# Autodesk Inventor assembly: YTP-AP-K01-R1.0
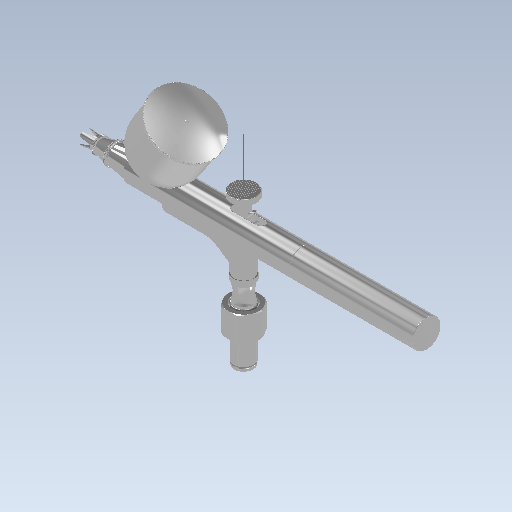
[picture p0: Inventor's stored thumbnail of the model, 512x512]
Saved by Autodesk Inventor 2020.4 (Build 244396000, 396)
## iProperties
RuleStatus: InUse
AfterDocNew0: iPropertyEnforcement
Created: 2021-08-29
Part Number: YTP-AP-K01-R1.0
Document SubType Name: Assembly
Designer: Uwe Wieser
Mass: 82.8737 g
Surface Area: 222.974 cm^2
Volume: 16.7279 cm^3
Density: 4.95421 g/cm^3
Project: Airbrush
Description: Iwata-HP-C-Airbrush
Author: Uwe Wieser
## Documents named in this file (23)
- F:\Autodesk-Inventor2020\YTP-Projekte\Airbrush\YTP-AP-K01-R1.0.iam
- F:\Autodesk-Inventor2020\YTP-Projekte\Airbrush\YTP-AP-E02-R1.0.ipt
- F:\Autodesk-Inventor2020\YTP-Projekte\Airbrush\YTP-AP-E03-R1.0.ipt
- F:\Autodesk-Inventor2020\YTP-Projekte\Airbrush\YTP-AP-E04-R1.0.ipt
- F:\Autodesk-Inventor2020\YTP-Projekte\Airbrush\YTP-AP-E05-R1.0.ipt
- F:\Autodesk-Inventor2020\YTP-Projekte\Airbrush\YTP-AP-E06-R1.0.ipt
- F:\Autodesk-Inventor2020\YTP-Projekte\Airbrush\YTP-AP-E07-R1.0.ipt
- F:\Autodesk-Inventor2020\YTP-Projekte\Airbrush\YTP-AP-E08-R1.0.ipt
- F:\Autodesk-Inventor2020\YTP-Projekte\Airbrush\YTP-AP-E09-R1.0.ipt
- F:\Autodesk-Inventor2020\YTP-Projekte\Airbrush\YTP-AP-E10-R1.0.ipt
- F:\Autodesk-Inventor2020\YTP-Projekte\Airbrush\YTP-AP-E11-R1.0.ipt
- F:\Autodesk-Inventor2020\YTP-Projekte\Airbrush\YTP-AP-E12-R1.0.ipt
- F:\Autodesk-Inventor2020\YTP-Projekte\Airbrush\YTP-AP-E13-R1.0.ipt
- F:\Autodesk-Inventor2020\YTP-Projekte\Airbrush\YTP-AP-E14-R1.0.ipt
- F:\Autodesk-Inventor2020\YTP-Projekte\Airbrush\YTP-AP-E15-R1.0.ipt
- F:\Autodesk-Inventor2020\YTP-Projekte\Airbrush\YTP-AP-E16-R1.0.ipt
- F:\Autodesk-Inventor2020\YTP-Projekte\Airbrush\YTP-AP-E17-R1.0.ipt
- F:\Autodesk-Inventor2020\YTP-Projekte\Airbrush\YTP-AP-E18-R1.0.ipt
- F:\Autodesk-Inventor2020\YTP-Projekte\Airbrush\YTP-AP-E19-R1.0.ipt
- F:\Autodesk-Inventor2020\YTP-Projekte\Airbrush\YTP-AP-E01-R1.1.ipt
- F:\Autodesk-Inventor2020\YTP-Projekte\Airbrush\YTP-AP-E20-R1.0.ipt
- F:\Autodesk-Inventor2020\YTP-Projekte\Airbrush\YTP-AP-E21-R1.0.ipt
- F:\Autodesk-Inventor2020\YTP-Projekte\Airbrush\YTP-AP-E22-R1.0.ipt
## Components (22 placed, 22 different names)
1. YTP-AP-E01-R1.1:1 — Passend:1, Fluchtend:1, Fluchtend:2, Einfügen:1, Passend:3, Tangential:1, Passend:4, Einfügen:2, Passend:6, Passend:7, Einfügen:5, Fluchtend:3, Einfügen:6, Fluchtend:4, Passend:16, Passend:17, Passend:20, Passend:27, Passend:28, Einfügen:7
2. YTP-AP-E02-R1.0:1 — Einfügen:2, Passend:7, Passend:19, Passend:21, Passend:25, Passend:30, Passend:31, Einfügen:9
3. YTP-AP-E03-R1.0:1 — Einfügen:1, Passend:29
4. YTP-AP-E04-R1.0:1 — Passend:2, Passend:3, Tangential:2
5. YTP-AP-E05-R1.0:1 — Passend:2, Tangential:1, Tangential:2
6. YTP-AP-E06-R1.0:1 — Passend:4, Passend:9, Passend:13, Passend:16
7. YTP-AP-E07-R1.0:1 — Einfügen:4, Passend:5, Passend:6, Einfügen:7
8. YTP-AP-E08-R1.0:1 — Einfügen:4, Passend:5
9. YTP-AP-E09-R1.0:1 — Einfügen:5, Passend:8
10. YTP-AP-E10-R1.0:1 — Fluchtend:3, Tangential:3, Passend:18, Tangential:4
11. YTP-AP-E11-R1.0:1 — Einfügen:6
12. YTP-AP-E12-R1.0:1 — Passend:9, Passend:10, Passend:11, Passend:12, Fluchtend:4
13. YTP-AP-E13-R1.0:1 — Passend:10, Passend:11, Passend:12, Passend:14, Winkel:1, Passend:15
14. YTP-AP-E14-R1.0:1 — Passend:13, Passend:14, Winkel:1, Passend:15, Passend:28, Einfügen:8
15. YTP-AP-E15-R1.0:2 — Tangential:3
16. YTP-AP-E16-R1.0:1 — Passend:21, Passend:24
17. YTP-AP-E17-R1.0:1 — Passend:19, Passend:20, Passend:23, Passend:26, Tangential:4
18. YTP-AP-E18-R1.0:1 — Passend:23, Passend:24, Passend:25
19. YTP-AP-E19-R1.0:1 — Passend:26, Passend:27
20. YTP-AP-E20-R1.0:1 — Passend:30, Passend:31
21. YTP-AP-E21-R1.0:1 — Einfügen:8
22. YTP-AP-E22-R1.0:1 — Einfügen:9
## Relationships (47: Mate 30, Insert 8, Flush 4, Tangent 4, Angle 1)
- Passend:1 [Mate]: YTP-AP-E01-R1.1:1
- Fluchtend:1 [Flush]: YTP-AP-E01-R1.1:1
- Fluchtend:2 [Flush]: YTP-AP-E01-R1.1:1
- Einfügen:1 [Insert]: YTP-AP-E01-R1.1:1 ↔ YTP-AP-E03-R1.0:1
- Passend:2 [Mate]: YTP-AP-E04-R1.0:1 ↔ YTP-AP-E05-R1.0:1
- Passend:3 [Mate]: YTP-AP-E01-R1.1:1 ↔ YTP-AP-E04-R1.0:1
- Tangential:1: YTP-AP-E01-R1.1:1 ↔ YTP-AP-E05-R1.0:1
- Tangential:2: YTP-AP-E04-R1.0:1 ↔ YTP-AP-E05-R1.0:1
- Passend:4 [Mate]: YTP-AP-E01-R1.1:1 ↔ YTP-AP-E06-R1.0:1
- Einfügen:2 [Insert]: YTP-AP-E01-R1.1:1 ↔ YTP-AP-E02-R1.0:1
- Einfügen:4 [Insert]: YTP-AP-E07-R1.0:1 ↔ YTP-AP-E08-R1.0:1
- Passend:5 [Mate]: YTP-AP-E07-R1.0:1 ↔ YTP-AP-E08-R1.0:1
- Passend:6 [Mate]: YTP-AP-E01-R1.1:1 ↔ YTP-AP-E07-R1.0:1
- Passend:7 [Mate]: YTP-AP-E01-R1.1:1 ↔ YTP-AP-E02-R1.0:1
- Einfügen:5 [Insert]: YTP-AP-E01-R1.1:1 ↔ YTP-AP-E09-R1.0:1
- Passend:8 [Mate]: YTP-AP-E09-R1.0:1
- Fluchtend:3 [Flush]: YTP-AP-E01-R1.1:1 ↔ YTP-AP-E10-R1.0:1
- Einfügen:6 [Insert]: YTP-AP-E01-R1.1:1 ↔ YTP-AP-E11-R1.0:1
- Passend:9 [Mate]: YTP-AP-E06-R1.0:1 ↔ YTP-AP-E12-R1.0:1
- Passend:10 [Mate]: YTP-AP-E12-R1.0:1 ↔ YTP-AP-E13-R1.0:1
- Passend:11 [Mate]: YTP-AP-E12-R1.0:1 ↔ YTP-AP-E13-R1.0:1
- Passend:12 [Mate]: YTP-AP-E12-R1.0:1 ↔ YTP-AP-E13-R1.0:1
- Passend:13 [Mate]: YTP-AP-E06-R1.0:1 ↔ YTP-AP-E14-R1.0:1
- Passend:14 [Mate]: YTP-AP-E13-R1.0:1 ↔ YTP-AP-E14-R1.0:1
- Winkel:1 [Angle] (0 deg): YTP-AP-E13-R1.0:1 ↔ YTP-AP-E14-R1.0:1
- Passend:15 [Mate]: YTP-AP-E13-R1.0:1 ↔ YTP-AP-E14-R1.0:1
- Fluchtend:4 [Flush] (8 mm): YTP-AP-E01-R1.1:1 ↔ YTP-AP-E12-R1.0:1
- Tangential:3: YTP-AP-E10-R1.0:1 ↔ YTP-AP-E15-R1.0:2
- Passend:16 [Mate]: YTP-AP-E01-R1.1:1 ↔ YTP-AP-E06-R1.0:1
- Passend:17 [Mate]: YTP-AP-E01-R1.1:1
- Passend:18 [Mate]: YTP-AP-E10-R1.0:1
- Passend:19 [Mate]: YTP-AP-E02-R1.0:1 ↔ YTP-AP-E17-R1.0:1
- Passend:20 [Mate]: YTP-AP-E01-R1.1:1 ↔ YTP-AP-E17-R1.0:1
- Passend:21 [Mate]: YTP-AP-E02-R1.0:1 ↔ YTP-AP-E16-R1.0:1
- Passend:23 [Mate]: YTP-AP-E17-R1.0:1 ↔ YTP-AP-E18-R1.0:1
- Passend:24 [Mate]: YTP-AP-E16-R1.0:1 ↔ YTP-AP-E18-R1.0:1
- Passend:25 [Mate]: YTP-AP-E02-R1.0:1 ↔ YTP-AP-E18-R1.0:1
- Passend:26 [Mate]: YTP-AP-E17-R1.0:1 ↔ YTP-AP-E19-R1.0:1
- Passend:27 [Mate]: YTP-AP-E01-R1.1:1 ↔ YTP-AP-E19-R1.0:1
- Tangential:4: YTP-AP-E10-R1.0:1 ↔ YTP-AP-E17-R1.0:1
- Passend:28 [Mate]: YTP-AP-E01-R1.1:1 ↔ YTP-AP-E14-R1.0:1
- Einfügen:7 [Insert]: YTP-AP-E01-R1.1:1 ↔ YTP-AP-E07-R1.0:1
- Passend:29 [Mate]: YTP-AP-E03-R1.0:1
- Passend:30 [Mate]: YTP-AP-E02-R1.0:1 ↔ YTP-AP-E20-R1.0:1
- Passend:31 [Mate]: YTP-AP-E02-R1.0:1 ↔ YTP-AP-E20-R1.0:1
- Einfügen:8 [Insert] (-2 mm): YTP-AP-E14-R1.0:1 ↔ YTP-AP-E21-R1.0:1
- Einfügen:9 [Insert]: YTP-AP-E02-R1.0:1 ↔ YTP-AP-E22-R1.0:1
